# Autodesk Inventor assembly: For Cabinet W=600
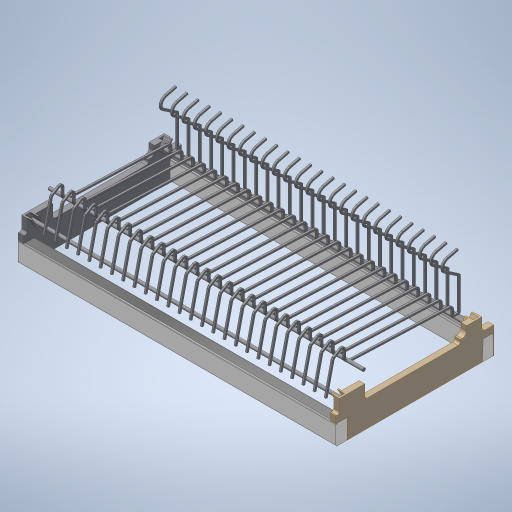
[picture p0: Inventor's stored thumbnail of the model, 512x512]
Saved by Autodesk Inventor 2024 (Build 280153000, 153)
## iProperties
RuleStatus: InUse
Created: 2017-01-23
Part Number: For Cabinet W=600
Document SubType Name: Assembly
Designer: SvetlanaB
Description: For Cabinet W=600
Author: SvetlanaB
## Documents named in this file (8)
- C:\W4INV 2024 Design\iBOX LIBRARY\Kitchen\Wall Cabinets\Dish Rack\Dish Rack Wire.iam
- C:\W4INV 2024 Design\iBOX LIBRARY\Kitchen\Wall Cabinets\Dish Rack\Right Dish Rack panel.ipt
- C:\W4INV 2024 Design\iBOX LIBRARY\Kitchen\Wall Cabinets\Dish Rack\Rod_1.ipt
- C:\W4INV 2024 Design\iBOX LIBRARY\Kitchen\Wall Cabinets\Dish Rack\Wire.ipt
- C:\W4INV 2024 Design\iBOX LIBRARY\Kitchen\Wall Cabinets\Dish Rack\Rod_2.ipt
- C:\W4INV 2024 Design\iBOX LIBRARY\Kitchen\Wall Cabinets\Dish Rack\Left Dish Rack panel_2.ipt
- C:\W4INV 2024 Design\iBOX LIBRARY\Kitchen\Wall Cabinets\Dish Rack\Frame.ipt
- C:\W4INV 2024 Design\iBOX LIBRARY\Kitchen\Wall Cabinets\Dish Rack\Dish Rack.ipt
## Components (8 placed, 7 different names)
1. @Skeleton — Flush:1, Flush:2, Flush:3
2. Right Dish Rack panel:1 — Mate:1
3. Rod_1:1
4. Wire:1
5. Rod_2:1
6. Rod_2:2 — Mate:1
7. Left Dish Rack panel_2:1
8. Frame:1
## Relationships (4: Flush 3, Mate 1)
- Mate:1: Right Dish Rack panel:1 ↔ Rod_2:2
- Flush:1: @Skeleton
- Flush:2: @Skeleton
- Flush:3: @Skeleton
